# Autodesk Inventor assembly: mount assem
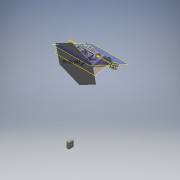
[picture p0: Inventor's stored thumbnail of the model, 180x180]
Saved by Autodesk Inventor 2019.3 (Build 233278000, 278)
## iProperties
Created: 2018-10-05
Part Number: mount assem
Document SubType Name: Assembly
Designer: HIVE
Author: HIVE
## Documents named in this file (6)
- D:\hive\projects\pocketpelvis\models\mounts\V2\femur\old stuff\mount assem.iam
- D:\hive\projects\pocketpelvis\models\mounts\V2\femur\old stuff\3945K300_HIGH-PULL RARE EARTH MAGNETIC BALL.ipt
- D:\hive\projects\pocketpelvis\models\mounts\V2\femur\old stuff\mounter.ipt
- D:\hive\projects\pocketpelvis\models\mounts\V2\Imported Components\pelvis_scaled1point6\pelvis_scaled1point6.ipt
- D:\hive\projects\pocketpelvis\models\mounts\V2\femur\shaft toothed clip toothed v2.ipt
- D:\hive\projects\pocketpelvis\models\mounts\V2\femur\shaft toothed.ipt
## Components (7 placed, 5 different names)
1. pelvis_scaled1point6:2
2. 3945K300_HIGH-PULL RARE EARTH MAGNETIC BALL:1 — Mate:3
3. 3945K300_HIGH-PULL RARE EARTH MAGNETIC BALL:2 — Mate:4
4. mounter:1 — Mate:8, Mate:10, Mate:11, Mate:15
5. shaft toothed clip toothed v2:1 — Mate:13
6. shaft toothed:1 — Mate:11
7. shaft toothed clip toothed v2:2 — Mate:15, Mate:16
## Relationships (11: Mate 10, Angle 1)
- Mate:3: 3945K300_HIGH-PULL RARE EARTH MAGNETIC BALL:1
- Mate:4: 3945K300_HIGH-PULL RARE EARTH MAGNETIC BALL:2
- Mate:5
- Mate:6
- Mate:8: mounter:1
- Mate:10: mounter:1
- Angle:1 (-155 deg)
- Mate:11: mounter:1 ↔ shaft toothed:1
- Mate:13: shaft toothed clip toothed v2:1
- Mate:15: mounter:1 ↔ shaft toothed clip toothed v2:2
- Mate:16: shaft toothed clip toothed v2:2
